# Autodesk Inventor assembly: Adjustable Elbow 1 Inch
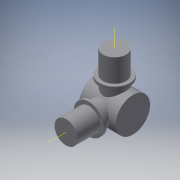
[picture p0: Inventor's stored thumbnail of the model, 180x180]
Saved by Autodesk Inventor 2018 (Build 220112000, 112)
## iProperties
Created: 2018-01-10
Part Number: Adjustable Elbow 1 Inch
Document SubType Name: Assembly
Designer: owner
Author: owner
## Documents named in this file (2)
- Z:\The Pickle\Inventor Pipe Parts\Formufit Fittings\Adjustable Elbow 1 Inch.iam
- Z:\The Pickle\Inventor Pipe Parts\Formufit Fittings\Adjustable Elbow\Adjustable elbow piece 1 inch.ipt
## Components (2 placed, 1 different names)
1. Adjustable elbow piece 1 inch:1 — Mate:1, Angle:1
2. Adjustable elbow piece 1 inch:2 — Mate:1, Angle:1
## Relationships (2: Mate 1, Angle 1)
- Mate:1: Adjustable elbow piece 1 inch:1 ↔ Adjustable elbow piece 1 inch:2
- Angle:1 (90 deg): Adjustable elbow piece 1 inch:1 ↔ Adjustable elbow piece 1 inch:2
